# Autodesk Inventor assembly: krmič
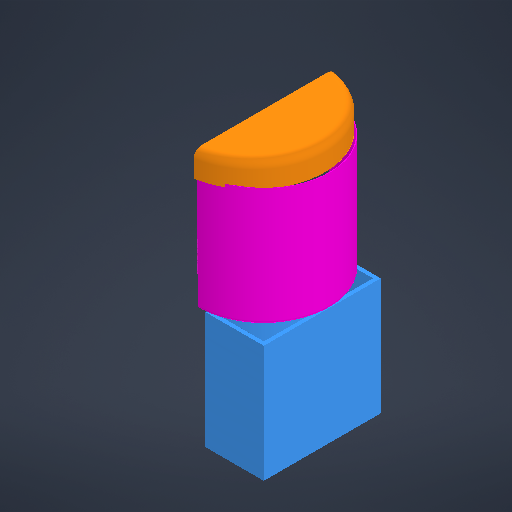
[picture p0: Inventor's stored thumbnail of the model, 512x512]
Saved by Autodesk Inventor 2026.2 (Build 302298000, 298)
## iProperties
Created: 2025-12-19
Part Number: krmič
Document SubType Name: Assembly
Designer: cerna
Author: cerna
## Documents named in this file (6)
- C:\Users\cerna\OneDrive\Plocha\Eliška\3D modely\krmič.iam
- C:\Users\cerna\OneDrive\Plocha\Eliška\3D modely\Box na elektrotechniku oprava.ipt
- C:\Users\cerna\OneDrive\Plocha\Eliška\3D modely\Naběračka.ipt
- C:\Users\cerna\OneDrive\Plocha\Eliška\3D modely\motor.ipt
- C:\Users\cerna\OneDrive\Plocha\Eliška\3D modely\Zásobník oprava.ipt
- C:\Users\cerna\OneDrive\Plocha\Eliška\3D modely\Poklop.ipt
## Components (5 placed, 5 different names)
1. Box na elektrotechniku oprava:1 — Stejný směr:1, Proti sobě:2, Proti sobě:3, Proti sobě:4, Proti sobě:5, Proti sobě:8, Proti sobě:13
2. Naběračka:1 — Proti sobě:6, Proti sobě:7
3. motor:1 — Proti sobě:4, Proti sobě:5, Proti sobě:6, Proti sobě:7, Proti sobě:8
4. Zásobník oprava:1 — Proti sobě:11, Proti sobě:12, Proti sobě:13, Stejný směr:15
5. Poklop:1 — Proti sobě:11, Proti sobě:12
## Relationships (12: Mate 10, Flush 2)
- Stejný směr:1 [Flush]: Box na elektrotechniku oprava:1
- Proti sobě:2 [Mate]: Box na elektrotechniku oprava:1
- Proti sobě:3 [Mate]: Box na elektrotechniku oprava:1
- Proti sobě:4 [Mate]: Box na elektrotechniku oprava:1 ↔ motor:1
- Proti sobě:5 [Mate]: Box na elektrotechniku oprava:1 ↔ motor:1
- Proti sobě:6 [Mate]: Naběračka:1 ↔ motor:1
- Proti sobě:7 [Mate]: Naběračka:1 ↔ motor:1
- Proti sobě:8 [Mate]: Box na elektrotechniku oprava:1 ↔ motor:1
- Proti sobě:11 [Mate]: Zásobník oprava:1 ↔ Poklop:1
- Proti sobě:12 [Mate]: Zásobník oprava:1 ↔ Poklop:1
- Proti sobě:13 [Mate]: Box na elektrotechniku oprava:1 ↔ Zásobník oprava:1
- Stejný směr:15 [Flush]: Zásobník oprava:1
